# Autodesk Inventor assembly: Ensamblaje3
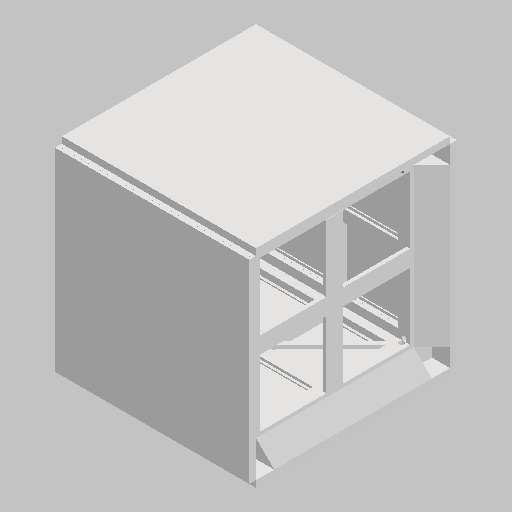
[picture p0: Inventor's stored thumbnail of the model, 512x512]
Saved by Autodesk Inventor 2027 (Build 310192000, 192)
## iProperties
Created: 2026-10-06
Part Number: Ensamblaje3
Document SubType Name: Assembly
Designer: Alexander
Author: Alexander
## Documents named in this file (4)
- C:\Users\Alexander\Documents\Digital Piezas\Ensamblaje3.iam
- C:\Users\Alexander\Documents\Digital Piezas\Frontal.ipt
- C:\Users\Alexander\Documents\Digital Piezas\MpoduloPanel;.ipt
- C:\Users\Alexander\Documents\Digital Piezas\EsctructuraCaja.ipt
## Components (9 placed, 3 different names)
1. Frontal:1 — De rotación:1
2. MpoduloPanel;:1 — De rotación:1, De rotación:4
3. EsctructuraCaja:1 — De rotación:4, Insertar:1, Insertar:2, Insertar:3, Insertar:4, Insertar:5
4. Frontal:2
5. MpoduloPanel;:2 — Insertar:1, Insertar:2
6. Frontal:3
7. MpoduloPanel;:3 — Insertar:3
8. Frontal:4
9. MpoduloPanel;:4 — Insertar:4, Insertar:5
## Relationships (10: RevoluteJoint 5, Insert 5)
- De rotación:1 [RevoluteJoint]: Frontal:1 ↔ MpoduloPanel;:1
- [RevoluteJoint]: Frontal:2 ↔ MpoduloPanel;:2
- [RevoluteJoint]: Frontal:3 ↔ MpoduloPanel;:3
- De rotación:4 [RevoluteJoint]: MpoduloPanel;:1 ↔ EsctructuraCaja:1
- [RevoluteJoint]: Frontal:4 ↔ MpoduloPanel;:4
- Insertar:1: EsctructuraCaja:1 ↔ MpoduloPanel;:2
- Insertar:2: EsctructuraCaja:1 ↔ MpoduloPanel;:2
- Insertar:3: EsctructuraCaja:1 ↔ MpoduloPanel;:3
- Insertar:4: EsctructuraCaja:1 ↔ MpoduloPanel;:4
- Insertar:5: EsctructuraCaja:1 ↔ MpoduloPanel;:4
## Named parameters: d4_d0 = 0 mm, d5_d1 = 270 deg, d6_d0 = 0 mm, d7_d1 = 270 deg, d12_d4_d0 = 0 mm, d13_d5_d1 = 270 deg
